# Autodesk Inventor assembly: Drivebase Assembly
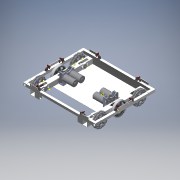
[picture p0: Inventor's stored thumbnail of the model, 180x180]
Saved by Autodesk Inventor 2018 (Build 220112000, 112)
## iProperties
Created: 2018-01-13
Part Number: Drivebase Assembly
Document SubType Name: Assembly
Designer: maste
Mass: 34303 g
Surface Area: 41903.7 cm^2
Volume: 33169.5 cm^3
Density: 1.03417 g/cm^3
Author: maste
## Documents named in this file (19)
- C:\Users\s-2512711\Downloads\Drivebase 2018 Files Final Kinda (5)\Drivebase 2018 Files Final Kinda\Drivebase 2018 Files Final Kinda\Drivebase 2018 Files 2\Drivebase 2018 Files 2\Drivebase Assembly.iam
- C:\Users\s-2512711\Downloads\Drivebase 2018 Files Final Kinda (5)\Drivebase 2018 Files Final Kinda\Drivebase 2018 Files Final Kinda\Drivebase 2018 Files 2\Drivebase 2018 Files 2\6in Wheel.iam
- C:\Users\s-2512711\Downloads\Drivebase 2018 Files Final Kinda (5)\Drivebase 2018 Files Final Kinda\Drivebase 2018 Files Final Kinda\Drivebase 2018 Files 2\Drivebase 2018 Files 2\BaseDrive\BaseDrive\BaseDrive Frame.iam
- C:\Users\s-2512711\Downloads\Drivebase 2018 Files Final Kinda (5)\Drivebase 2018 Files Final Kinda\Drivebase 2018 Files Final Kinda\Drivebase 2018 Files 2\Drivebase 2018 Files 2\new_folder__2_\New folder (2)\2x2x26.ipt
- C:\Users\s-2512711\Downloads\Drivebase 2018 Files Final Kinda (5)\Drivebase 2018 Files Final Kinda\Drivebase 2018 Files Final Kinda\Drivebase 2018 Files 2\Drivebase 2018 Files 2\new_folder__2_\New folder (2)\1x2x23.ipt
- C:\Users\s-2512711\Downloads\Drivebase 2018 Files Final Kinda (5)\Drivebase 2018 Files Final Kinda\Drivebase 2018 Files Final Kinda\Drivebase 2018 Files 2\Drivebase 2018 Files 2\new_folder__2_\New folder (2)\1x2x2.ipt
- C:\Users\s-2512711\Downloads\Drivebase 2018 Files Final Kinda (5)\Drivebase 2018 Files Final Kinda\Drivebase 2018 Files Final Kinda\Drivebase 2018 Files 2\Drivebase 2018 Files 2\0_500_Hex_ID_x_1_125_OD_x_0_313_WD_Flanged_Bearing_v2_217-3875.ipt
- C:\Users\s-2512711\Downloads\Drivebase 2018 Files Final Kinda (5)\Drivebase 2018 Files Final Kinda\Drivebase 2018 Files Final Kinda\Drivebase 2018 Files 2\Drivebase 2018 Files 2\Pulley.iam
- C:\Users\s-2512711\Downloads\Drivebase 2018 Files Final Kinda (5)\Drivebase 2018 Files Final Kinda\Drivebase 2018 Files Final Kinda\Drivebase 2018 Files 2\Drivebase 2018 Files 2\Gearbox.iam
- C:\Users\s-2512711\Downloads\Drivebase 2018 Files Final Kinda (5)\Drivebase 2018 Files Final Kinda\Drivebase 2018 Files Final Kinda\Drivebase 2018 Files 2\Drivebase 2018 Files 2\3in hex shaft.ipt
- C:\Users\s-2512711\Downloads\Drivebase 2018 Files Final Kinda (5)\Drivebase 2018 Files Final Kinda\Drivebase 2018 Files Final Kinda\Drivebase 2018 Files 2\Drivebase 2018 Files 2\36t_x_9mm_Wide_Double_Flange_Aluminum_Pulley_GT2_3mm_1_2_Hex_Bore_217-5873.ipt
- C:\Users\s-2512711\Downloads\Drivebase 2018 Files Final Kinda (5)\Drivebase 2018 Files Final Kinda\Drivebase 2018 Files Final Kinda\Drivebase 2018 Files 2\Drivebase 2018 Files 2\Omni Wheel.iam
- C:\Users\s-2512711\Downloads\Drivebase 2018 Files Final Kinda (5)\Drivebase 2018 Files Final Kinda\Drivebase 2018 Files Final Kinda\Drivebase 2018 Files 2\Drivebase 2018 Files 2\L gusset.ipt
- C:\Users\s-2512711\Downloads\Drivebase 2018 Files Final Kinda (5)\Drivebase 2018 Files Final Kinda\Drivebase 2018 Files Final Kinda\Drivebase 2018 Files 2\Drivebase 2018 Files 2\4461-17-0101 + Bearing.iam
- C:\Users\s-2512711\Downloads\Drivebase 2018 Files Final Kinda (5)\Drivebase 2018 Files Final Kinda\Drivebase 2018 Files Final Kinda\Drivebase 2018 Files 2\Drivebase 2018 Files 2\L Bracket 3in.ipt
- C:\Users\s-2512711\Downloads\Drivebase 2018 Files Final Kinda (5)\Drivebase 2018 Files Final Kinda\Drivebase 2018 Files Final Kinda\Drivebase 2018 Files 2\Drivebase 2018 Files 2\L Bracket 4in.ipt
- C:\Users\s-2512711\Downloads\Drivebase 2018 Files Final Kinda (5)\Drivebase 2018 Files Final Kinda\Drivebase 2018 Files Final Kinda\Drivebase 2018 Files 2\Drivebase 2018 Files 2\L Bracket 6in.ipt
- C:\Users\s-2512711\Downloads\Drivebase 2018 Files Final Kinda (5)\Drivebase 2018 Files Final Kinda\Drivebase 2018 Files Final Kinda\Drivebase 2018 Files 2\Drivebase 2018 Files 2\Bumper.ipt
- C:\Users\s-2512711\Downloads\Drivebase 2018 Files Final Kinda (5)\Drivebase 2018 Files Final Kinda\Drivebase 2018 Files Final Kinda\Drivebase 2018 Files 2\Drivebase 2018 Files 2\Belly Pan.ipt
## Components (52 placed, 18 different names)
1. 6in Wheel:1 [sub-assembly] — Mate:107, Mate:108, Mate:109, Rotation:8
2. 6in Wheel:2 [sub-assembly] — Mate:116, Mate:117, Mate:118, Rotation:11
3. BaseDrive Frame:1 [sub-assembly] — Mate:207, Mate:208, Mate:209, Mate:210, Mate:211, Mate:212, Mate:213, Mate:214, Mate:215, Mate:216, Mate:217, Mate:218, Mate:232, Mate:233, Mate:234, Mate:235, Mate:236, Mate:237, Mate:238, Mate:239, Mate:240, Mate:241, Mate:242, Mate:243, Mate:270, Mate:271, Mate:287, Mate:354, Mate:355, Mate:360, Mate:361, Mate:363, Mate:383, Mate:384, Mate:385, Mate:390, Mate:391
4. 2x2x26:1 — Mate:93, Rotation:1, Mate:94, Mate:95, Rotation:2, Mate:151, Mate:220, Mate:250, Mate:251, Mate:252, Mate:253, Mate:254, Mate:255, Mate:288, Mate:291, Mate:296, Mate:297, Mate:298, Mate:304, Mate:327, Mate:328, Mate:331, Mate:332, Mate:333, Mate:338, Mate:376, Mate:394
5. 2x2x26:2 — Mate:100, Mate:101, Rotation:5, Mate:244, Mate:245, Mate:246, Mate:247, Mate:248, Mate:249, Mate:292, Mate:293, Mate:294, Mate:295, Mate:299, Mate:300, Mate:310, Mate:311, Mate:312, Mate:378, Mate:386
6. 1x2x23:1 — Mate:294, Mate:295, Mate:374, Mate:375, Mate:383
7. 1x2x2:1 — Mate:287, Mate:288, Mate:291, Mate:384
8. 1x2x2:2 — Mate:292, Mate:293, Mate:385
9. 0_500_Hex_ID_x_1_125_OD_x_0_313_WD_Flanged_Bearing_v2_217-3875:2 — Mate:100, Mate:101, Rotation:5, Mate:116, Mate:117, Mate:118, Rotation:11, Mate:158
10. 0_500_Hex_ID_x_1_125_OD_x_0_313_WD_Flanged_Bearing_v2_217-3875:5 — Mate:94, Mate:95, Rotation:2, Mate:107, Mate:108, Mate:109, Rotation:8, Mate:150
11. 0_500_Hex_ID_x_1_125_OD_x_0_313_WD_Flanged_Bearing_v2_217-3875:6 — Mate:93, Rotation:1, Mate:220, Mate:325, Mate:373
12. Pulley:1 [sub-assembly] — Mate:324, Mate:325, Mate:346, Mate:347, Mate:348, Mate:373
13. Pulley:4 [sub-assembly] — Mate:319, Mate:379, Mate:380, Mate:387, Mate:388
14. Gearbox:1 [sub-assembly] — Mate:143, Mate:144, Mate:148, Mate:149, Mate:296, Mate:297, Mate:298, Mate:394
15. Gearbox:2 [sub-assembly] — Mate:155, Mate:156, Mate:157, Mate:162, Mate:163, Mate:164, Mate:299, Mate:300
16. 3in hex shaft:1 — Mate:334, Mate:335, Mate:336, Mate:337, Mate:350, Mate:351
17. 3in hex shaft:2 — Mate:339, Mate:340, Mate:341, Mate:342, Mate:343, Mate:371, Mate:372
18. 36t_x_9mm_Wide_Double_Flange_Aluminum_Pulley_GT2_3mm_1_2_Hex_Bore_217-5873:1 — Mate:336, Mate:337, Mate:338
19. 36t_x_9mm_Wide_Double_Flange_Aluminum_Pulley_GT2_3mm_1_2_Hex_Bore_217-5873:2 — Mate:370, Mate:371, Mate:372
20. 36t_x_9mm_Wide_Double_Flange_Aluminum_Pulley_GT2_3mm_1_2_Hex_Bore_217-5873:3 — Mate:155, Mate:156, Mate:157, Mate:158
21. 36t_x_9mm_Wide_Double_Flange_Aluminum_Pulley_GT2_3mm_1_2_Hex_Bore_217-5873:4 — Mate:162, Mate:163, Mate:164
22. 36t_x_9mm_Wide_Double_Flange_Aluminum_Pulley_GT2_3mm_1_2_Hex_Bore_217-5873:5 — Mate:143, Mate:144, Mate:151
23. 36t_x_9mm_Wide_Double_Flange_Aluminum_Pulley_GT2_3mm_1_2_Hex_Bore_217-5873:6 — Mate:148, Mate:149, Mate:150
24. L gusset:1 — Mate:216, Mate:217, Mate:218
25. L gusset:2 — Mate:213, Mate:214, Mate:215
26. L gusset:3 — Mate:210, Mate:211, Mate:212
27. L gusset:4 — Mate:207, Mate:208, Mate:209
28. L gusset:5 — Mate:235, Mate:236, Mate:237, Mate:362
29. L gusset:6 — Mate:238, Mate:239, Mate:240, Mate:359
30. L gusset:7 — Mate:241, Mate:242, Mate:243, Mate:353
31. L gusset:8 — Mate:232, Mate:233, Mate:234, Mate:356
32. 4461-17-0101 + Bearing:1 [sub-assembly] — Mate:253, Mate:254, Mate:255, Mate:304, Rotation:12, Mate:334, Mate:335
33. 4461-17-0101 + Bearing:2 [sub-assembly] — Mate:250, Mate:251, Mate:252, Mate:324
34. 4461-17-0101 + Bearing:3 [sub-assembly] — Mate:247, Mate:248, Mate:249, Mate:319, Flush:1, Mate:379, Mate:380
35. 4461-17-0101 + Bearing:4 [sub-assembly] — Mate:244, Mate:245, Mate:246, Mate:339, Mate:340, Mate:341
36. L Bracket 3in:1 — Mate:353, Mate:354, Mate:355
37. L Bracket 3in:2 — Mate:356
38. L Bracket 4in:1 — Mate:359, Mate:360, Mate:361, Mate:377
39. L Bracket 4in:2 — Mate:362, Mate:363, Mate:393
40. L Bracket 6in:1 — Mate:270, Mate:271, Mate:277, Mate:281
41. L Bracket 6in:2 — Mate:283, Mate:284, Mate:390, Mate:391, Mate:392
42. Bumper:1 — Mate:277, Mate:281, Mate:377
43. Bumper:2 — Mate:283, Mate:284, Mate:392, Mate:393
44. Omni Wheel:1 [sub-assembly] — Mate:347, Mate:348, Mate:349
45. Omni Wheel:2 [sub-assembly] — Mate:342, Mate:343, Mate:344
46. Omni Wheel:3 [sub-assembly] — Mate:387, Mate:388, Mate:389
47. Omni Wheel:4 [sub-assembly] — Mate:350, Mate:351, Mate:352
48. 4461-17-0101 + Bearing:5 [sub-assembly] — Flush:1, Mate:378, Mate:386, Mate:389
49. 4461-17-0101 + Bearing:6 [sub-assembly] — Mate:310, Mate:311, Mate:312, Mate:344, Mate:370
50. 4461-17-0101 + Bearing:7 [sub-assembly] — Mate:327, Mate:328, Mate:346, Mate:349
51. 4461-17-0101 + Bearing:8 [sub-assembly] — Mate:331, Mate:332, Mate:333, Rotation:12, Mate:352
52. Belly Pan:1 — Mate:374, Mate:375, Mate:376
## Relationships (148: Mate 141, RelateRotation 6, Flush 1)
- Mate:93: 2x2x26:1 ↔ 0_500_Hex_ID_x_1_125_OD_x_0_313_WD_Flanged_Bearing_v2_217-3875:6
- Rotation:1 [RelateRotation] (1 ul): 2x2x26:1 ↔ 0_500_Hex_ID_x_1_125_OD_x_0_313_WD_Flanged_Bearing_v2_217-3875:6
- Mate:94: 2x2x26:1 ↔ 0_500_Hex_ID_x_1_125_OD_x_0_313_WD_Flanged_Bearing_v2_217-3875:5
- Mate:95: 2x2x26:1 ↔ 0_500_Hex_ID_x_1_125_OD_x_0_313_WD_Flanged_Bearing_v2_217-3875:5
- Rotation:2 [RelateRotation] (1 ul): 2x2x26:1 ↔ 0_500_Hex_ID_x_1_125_OD_x_0_313_WD_Flanged_Bearing_v2_217-3875:5
- Mate:100: 2x2x26:2 ↔ 0_500_Hex_ID_x_1_125_OD_x_0_313_WD_Flanged_Bearing_v2_217-3875:2
- Mate:101: 2x2x26:2 ↔ 0_500_Hex_ID_x_1_125_OD_x_0_313_WD_Flanged_Bearing_v2_217-3875:2
- Rotation:5 [RelateRotation] (1 ul): 2x2x26:2 ↔ 0_500_Hex_ID_x_1_125_OD_x_0_313_WD_Flanged_Bearing_v2_217-3875:2
- Mate:107: 6in Wheel:1 ↔ 0_500_Hex_ID_x_1_125_OD_x_0_313_WD_Flanged_Bearing_v2_217-3875:5
- Mate:108: 6in Wheel:1 ↔ 0_500_Hex_ID_x_1_125_OD_x_0_313_WD_Flanged_Bearing_v2_217-3875:5
- Mate:109: 6in Wheel:1 ↔ 0_500_Hex_ID_x_1_125_OD_x_0_313_WD_Flanged_Bearing_v2_217-3875:5
- Rotation:8 [RelateRotation] (1 ul): 6in Wheel:1 ↔ 0_500_Hex_ID_x_1_125_OD_x_0_313_WD_Flanged_Bearing_v2_217-3875:5
- Mate:116: 6in Wheel:2 ↔ 0_500_Hex_ID_x_1_125_OD_x_0_313_WD_Flanged_Bearing_v2_217-3875:2
- Mate:117: 6in Wheel:2 ↔ 0_500_Hex_ID_x_1_125_OD_x_0_313_WD_Flanged_Bearing_v2_217-3875:2
- Mate:118: 6in Wheel:2 ↔ 0_500_Hex_ID_x_1_125_OD_x_0_313_WD_Flanged_Bearing_v2_217-3875:2
- Rotation:11 [RelateRotation] (1 ul): 6in Wheel:2 ↔ 0_500_Hex_ID_x_1_125_OD_x_0_313_WD_Flanged_Bearing_v2_217-3875:2
- Mate:143: Gearbox:1 ↔ 36t_x_9mm_Wide_Double_Flange_Aluminum_Pulley_GT2_3mm_1_2_Hex_Bore_217-5873:5
- Mate:144: Gearbox:1 ↔ 36t_x_9mm_Wide_Double_Flange_Aluminum_Pulley_GT2_3mm_1_2_Hex_Bore_217-5873:5
- Mate:148: Gearbox:1 ↔ 36t_x_9mm_Wide_Double_Flange_Aluminum_Pulley_GT2_3mm_1_2_Hex_Bore_217-5873:6
- Mate:149: Gearbox:1 ↔ 36t_x_9mm_Wide_Double_Flange_Aluminum_Pulley_GT2_3mm_1_2_Hex_Bore_217-5873:6
- Mate:150: 0_500_Hex_ID_x_1_125_OD_x_0_313_WD_Flanged_Bearing_v2_217-3875:5 ↔ 36t_x_9mm_Wide_Double_Flange_Aluminum_Pulley_GT2_3mm_1_2_Hex_Bore_217-5873:6
- Mate:151: 2x2x26:1 ↔ 36t_x_9mm_Wide_Double_Flange_Aluminum_Pulley_GT2_3mm_1_2_Hex_Bore_217-5873:5
- Mate:155: Gearbox:2 ↔ 36t_x_9mm_Wide_Double_Flange_Aluminum_Pulley_GT2_3mm_1_2_Hex_Bore_217-5873:3
- Mate:156: Gearbox:2 ↔ 36t_x_9mm_Wide_Double_Flange_Aluminum_Pulley_GT2_3mm_1_2_Hex_Bore_217-5873:3
- Mate:157: Gearbox:2 ↔ 36t_x_9mm_Wide_Double_Flange_Aluminum_Pulley_GT2_3mm_1_2_Hex_Bore_217-5873:3
- Mate:158: 0_500_Hex_ID_x_1_125_OD_x_0_313_WD_Flanged_Bearing_v2_217-3875:2 ↔ 36t_x_9mm_Wide_Double_Flange_Aluminum_Pulley_GT2_3mm_1_2_Hex_Bore_217-5873:3
- Mate:162: Gearbox:2 ↔ 36t_x_9mm_Wide_Double_Flange_Aluminum_Pulley_GT2_3mm_1_2_Hex_Bore_217-5873:4
- Mate:163: Gearbox:2 ↔ 36t_x_9mm_Wide_Double_Flange_Aluminum_Pulley_GT2_3mm_1_2_Hex_Bore_217-5873:4
- Mate:164: Gearbox:2 ↔ 36t_x_9mm_Wide_Double_Flange_Aluminum_Pulley_GT2_3mm_1_2_Hex_Bore_217-5873:4
- Mate:207: BaseDrive Frame:1 ↔ L gusset:4
- Mate:208: BaseDrive Frame:1 ↔ L gusset:4
- Mate:209: BaseDrive Frame:1 ↔ L gusset:4
- Mate:210: BaseDrive Frame:1 ↔ L gusset:3
- Mate:211: BaseDrive Frame:1 ↔ L gusset:3
- Mate:212: BaseDrive Frame:1 ↔ L gusset:3
- Mate:213: BaseDrive Frame:1 ↔ L gusset:2
- Mate:214: BaseDrive Frame:1 ↔ L gusset:2
- Mate:215: BaseDrive Frame:1 ↔ L gusset:2
- Mate:216: BaseDrive Frame:1 ↔ L gusset:1
- Mate:217: BaseDrive Frame:1 ↔ L gusset:1
- Mate:218: BaseDrive Frame:1 ↔ L gusset:1
- Mate:220: 2x2x26:1 ↔ 0_500_Hex_ID_x_1_125_OD_x_0_313_WD_Flanged_Bearing_v2_217-3875:6
- Mate:232: BaseDrive Frame:1 ↔ L gusset:8
- Mate:233: BaseDrive Frame:1 ↔ L gusset:8
- Mate:234: BaseDrive Frame:1 ↔ L gusset:8
- Mate:235: BaseDrive Frame:1 ↔ L gusset:5
- Mate:236: BaseDrive Frame:1 ↔ L gusset:5
- Mate:237: BaseDrive Frame:1 ↔ L gusset:5
- Mate:238: BaseDrive Frame:1 ↔ L gusset:6
- Mate:239: BaseDrive Frame:1 ↔ L gusset:6
- Mate:240: BaseDrive Frame:1 ↔ L gusset:6
- Mate:241: BaseDrive Frame:1 ↔ L gusset:7
- Mate:242: BaseDrive Frame:1 ↔ L gusset:7
- Mate:243: BaseDrive Frame:1 ↔ L gusset:7
- Mate:244: 2x2x26:2 ↔ 4461-17-0101 + Bearing:4
- Mate:245: 2x2x26:2 ↔ 4461-17-0101 + Bearing:4
- Mate:246: 2x2x26:2 ↔ 4461-17-0101 + Bearing:4
- Mate:247: 2x2x26:2 ↔ 4461-17-0101 + Bearing:3
- Mate:248: 2x2x26:2 ↔ 4461-17-0101 + Bearing:3
- Mate:249: 2x2x26:2 ↔ 4461-17-0101 + Bearing:3
- Mate:250: 2x2x26:1 ↔ 4461-17-0101 + Bearing:2
- Mate:251: 2x2x26:1 ↔ 4461-17-0101 + Bearing:2
- Mate:252: 2x2x26:1 ↔ 4461-17-0101 + Bearing:2
- Mate:253: 2x2x26:1 ↔ 4461-17-0101 + Bearing:1
- Mate:254: 2x2x26:1 ↔ 4461-17-0101 + Bearing:1
- Mate:255: 2x2x26:1 ↔ 4461-17-0101 + Bearing:1
- Mate:270: BaseDrive Frame:1 ↔ L Bracket 6in:1
- Mate:271: BaseDrive Frame:1 ↔ L Bracket 6in:1
- Mate:277: L Bracket 6in:1 ↔ Bumper:1
- Mate:281: L Bracket 6in:1 ↔ Bumper:1
- Mate:283: L Bracket 6in:2 ↔ Bumper:2
- Mate:284: L Bracket 6in:2 ↔ Bumper:2
- Mate:287: BaseDrive Frame:1 ↔ 1x2x2:1
- Mate:288: 2x2x26:1 ↔ 1x2x2:1
- Mate:291: 2x2x26:1 ↔ 1x2x2:1
- Mate:292: 2x2x26:2 ↔ 1x2x2:2
- Mate:293: 2x2x26:2 ↔ 1x2x2:2
- Mate:294: 2x2x26:2 ↔ 1x2x23:1
- Mate:295: 2x2x26:2 ↔ 1x2x23:1
- Mate:296: 2x2x26:1 ↔ Gearbox:1
- Mate:297: 2x2x26:1 ↔ Gearbox:1
- Mate:298: 2x2x26:1 ↔ Gearbox:1
- Mate:299: 2x2x26:2 ↔ Gearbox:2
- Mate:300: 2x2x26:2 ↔ Gearbox:2
- Mate:304: 2x2x26:1 ↔ 4461-17-0101 + Bearing:1
- Mate:310: 2x2x26:2 ↔ 4461-17-0101 + Bearing:6
- Mate:311: 2x2x26:2 ↔ 4461-17-0101 + Bearing:6
- Mate:312: 2x2x26:2 ↔ 4461-17-0101 + Bearing:6
- Mate:319: Pulley:4 ↔ 4461-17-0101 + Bearing:3
- Mate:324: Pulley:1 ↔ 4461-17-0101 + Bearing:2
- Mate:325: 0_500_Hex_ID_x_1_125_OD_x_0_313_WD_Flanged_Bearing_v2_217-3875:6 ↔ Pulley:1
- Mate:327: 2x2x26:1 ↔ 4461-17-0101 + Bearing:7
- Mate:328: 2x2x26:1 ↔ 4461-17-0101 + Bearing:7
- Mate:331: 2x2x26:1 ↔ 4461-17-0101 + Bearing:8
- Mate:332: 2x2x26:1 ↔ 4461-17-0101 + Bearing:8
- Mate:333: 2x2x26:1 ↔ 4461-17-0101 + Bearing:8
- Rotation:12 [RelateRotation] (1 ul): 4461-17-0101 + Bearing:1 ↔ 4461-17-0101 + Bearing:8
- Mate:334: 3in hex shaft:1 ↔ 4461-17-0101 + Bearing:1
- Mate:335: 3in hex shaft:1 ↔ 4461-17-0101 + Bearing:1
- Mate:336: 3in hex shaft:1 ↔ 36t_x_9mm_Wide_Double_Flange_Aluminum_Pulley_GT2_3mm_1_2_Hex_Bore_217-5873:1
- Mate:337: 3in hex shaft:1 ↔ 36t_x_9mm_Wide_Double_Flange_Aluminum_Pulley_GT2_3mm_1_2_Hex_Bore_217-5873:1
- Mate:338: 2x2x26:1 ↔ 36t_x_9mm_Wide_Double_Flange_Aluminum_Pulley_GT2_3mm_1_2_Hex_Bore_217-5873:1
- Mate:339: 3in hex shaft:2 ↔ 4461-17-0101 + Bearing:4
- Mate:340: 3in hex shaft:2 ↔ 4461-17-0101 + Bearing:4
- Mate:341: 3in hex shaft:2 ↔ 4461-17-0101 + Bearing:4
- Mate:342: 3in hex shaft:2 ↔ Omni Wheel:2
- Mate:343: 3in hex shaft:2 ↔ Omni Wheel:2
- Mate:344: Omni Wheel:2 ↔ 4461-17-0101 + Bearing:6
- Mate:346: Pulley:1 ↔ 4461-17-0101 + Bearing:7
- Mate:347: Pulley:1 ↔ Omni Wheel:1
- Mate:348: Pulley:1 ↔ Omni Wheel:1
- Mate:349: Omni Wheel:1 ↔ 4461-17-0101 + Bearing:7
- Mate:350: 3in hex shaft:1 ↔ Omni Wheel:4
- Mate:351: 3in hex shaft:1 ↔ Omni Wheel:4
- Mate:352: Omni Wheel:4 ↔ 4461-17-0101 + Bearing:8
- Mate:353: L gusset:7 ↔ L Bracket 3in:1
- Mate:354: BaseDrive Frame:1 ↔ L Bracket 3in:1
- Mate:355: BaseDrive Frame:1 ↔ L Bracket 3in:1
- Mate:356: L gusset:8 ↔ L Bracket 3in:2
- Mate:359: L gusset:6 ↔ L Bracket 4in:1
- Mate:360: BaseDrive Frame:1 ↔ L Bracket 4in:1
- Mate:361: BaseDrive Frame:1 ↔ L Bracket 4in:1
- Mate:362: L gusset:5 ↔ L Bracket 4in:2
- Mate:363: BaseDrive Frame:1 ↔ L Bracket 4in:2
- Flush:1: 4461-17-0101 + Bearing:3 ↔ 4461-17-0101 + Bearing:5
- Mate:370: 36t_x_9mm_Wide_Double_Flange_Aluminum_Pulley_GT2_3mm_1_2_Hex_Bore_217-5873:2 ↔ 4461-17-0101 + Bearing:6
- Mate:371: 3in hex shaft:2 ↔ 36t_x_9mm_Wide_Double_Flange_Aluminum_Pulley_GT2_3mm_1_2_Hex_Bore_217-5873:2
- Mate:372: 3in hex shaft:2 ↔ 36t_x_9mm_Wide_Double_Flange_Aluminum_Pulley_GT2_3mm_1_2_Hex_Bore_217-5873:2
- Mate:373: 0_500_Hex_ID_x_1_125_OD_x_0_313_WD_Flanged_Bearing_v2_217-3875:6 ↔ Pulley:1
- Mate:374: 1x2x23:1 ↔ Belly Pan:1
- Mate:375: 1x2x23:1 ↔ Belly Pan:1
- Mate:376: 2x2x26:1 ↔ Belly Pan:1
- Mate:377: L Bracket 4in:1 ↔ Bumper:1
- Mate:378: 2x2x26:2 ↔ 4461-17-0101 + Bearing:5
- Mate:379: Pulley:4 ↔ 4461-17-0101 + Bearing:3
- Mate:380: Pulley:4 ↔ 4461-17-0101 + Bearing:3
- Mate:383: BaseDrive Frame:1 ↔ 1x2x23:1
- Mate:384: BaseDrive Frame:1 ↔ 1x2x2:1
- Mate:385: BaseDrive Frame:1 ↔ 1x2x2:2
- Mate:386: 2x2x26:2 ↔ 4461-17-0101 + Bearing:5
- Mate:387: Pulley:4 ↔ Omni Wheel:3
- Mate:388: Pulley:4 ↔ Omni Wheel:3
- Mate:389: Omni Wheel:3 ↔ 4461-17-0101 + Bearing:5
- Mate:390: BaseDrive Frame:1 ↔ L Bracket 6in:2
- Mate:391: BaseDrive Frame:1 ↔ L Bracket 6in:2
- Mate:392: L Bracket 6in:2 ↔ Bumper:2
- Mate:393: L Bracket 4in:2 ↔ Bumper:2
- Mate:394: 2x2x26:1 ↔ Gearbox:1
